# Autodesk Inventor assembly: Roller-ver4-1111-2021
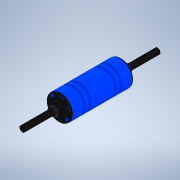
[picture p0: Inventor's stored thumbnail of the model, 180x180]
Saved by Autodesk Inventor 2021 (Build 250183000, 183)
## iProperties
Created: 2021-01-26
Part Number: Roller-ver4-1111-2021
Document SubType Name: Assembly
Designer: Caitlin
Author: Caitlin
## Documents named in this file (5)
- C:\Users\con_c_000\Documents\GitHub\RoboticsCad1111\PHRC CADD\2020 Infinite Recharge\2021 Infinite Recharge\Chassis\Roller-ver4-1111-2021.iam
- C:\Users\con_c_000\Documents\GitHub\RoboticsCad1111\PHRC CADD\2020 Infinite Recharge\Storage\Parts\Roller-ver3-1111-2019.ipt
- C:\Users\con_c_000\Documents\GitHub\RoboticsCad1111\PHRC CADD\Resources\VEXpro Resources\Versa Motion\VersaHub(0.5inHex)-1111-2016.ipt
- C:\Users\con_c_000\Documents\GitHub\RoboticsCad1111\PHRC CADD\Resources\VEXpro Resources\Spacers\0.25inAcetalSpacer(0.5inHex)-1111-2016.ipt
- C:\Users\con_c_000\Documents\GitHub\RoboticsCad1111\PHRC CADD\2020 Infinite Recharge\2021 Infinite Recharge\Chassis\0.5inThunderHexShaft(12in))-1111-2021.ipt
## Components (6 placed, 4 different names)
1. Roller-ver3-1111-2019:2 — Rotational:1, Rotational:2, Flush:1
2. VersaHub(0.5inHex)-1111-2016:3 — Rotational:1, Mate:2, Cylindrical:1, Angle:1
3. VersaHub(0.5inHex)-1111-2016:4 — Rotational:2, Mate:1, Angle:2
4. 0.25inAcetalSpacer(0.5inHex)-1111-2016:1 — Mate:1, Cylindrical:4, Angle:5
5. 0.25inAcetalSpacer(0.5inHex)-1111-2016:2 — Mate:2, Cylindrical:2, Angle:3
6. 0.5inThunderHexShaft(12in))-1111-2021:1 — Cylindrical:1, Flush:1, Angle:1, Angle:2, Cylindrical:2, Angle:3, Cylindrical:4, Angle:5
## Relationships (12: Angle 4, CylindricalJoint 3, RevoluteJoint 2, Mate 2, Flush 1)
- Rotational:1 [RevoluteJoint]: Roller-ver3-1111-2019:2 ↔ VersaHub(0.5inHex)-1111-2016:3
- Rotational:2 [RevoluteJoint]: Roller-ver3-1111-2019:2 ↔ VersaHub(0.5inHex)-1111-2016:4
- Mate:1: VersaHub(0.5inHex)-1111-2016:4 ↔ 0.25inAcetalSpacer(0.5inHex)-1111-2016:1
- Mate:2: VersaHub(0.5inHex)-1111-2016:3 ↔ 0.25inAcetalSpacer(0.5inHex)-1111-2016:2
- Cylindrical:1: VersaHub(0.5inHex)-1111-2016:3 ↔ 0.5inThunderHexShaft(12in))-1111-2021:1
- Flush:1 (85.725 mm): Roller-ver3-1111-2019:2 ↔ 0.5inThunderHexShaft(12in))-1111-2021:1
- Angle:1 (90 deg): VersaHub(0.5inHex)-1111-2016:3 ↔ 0.5inThunderHexShaft(12in))-1111-2021:1
- Angle:2 (90 deg): VersaHub(0.5inHex)-1111-2016:4 ↔ 0.5inThunderHexShaft(12in))-1111-2021:1
- Cylindrical:2: 0.25inAcetalSpacer(0.5inHex)-1111-2016:2 ↔ 0.5inThunderHexShaft(12in))-1111-2021:1
- Angle:3 (90 deg): 0.25inAcetalSpacer(0.5inHex)-1111-2016:2 ↔ 0.5inThunderHexShaft(12in))-1111-2021:1
- Cylindrical:4: 0.25inAcetalSpacer(0.5inHex)-1111-2016:1 ↔ 0.5inThunderHexShaft(12in))-1111-2021:1
- Angle:5 (90 deg): 0.25inAcetalSpacer(0.5inHex)-1111-2016:1 ↔ 0.5inThunderHexShaft(12in))-1111-2021:1
